# Autodesk Inventor assembly: аккумулятор 18650
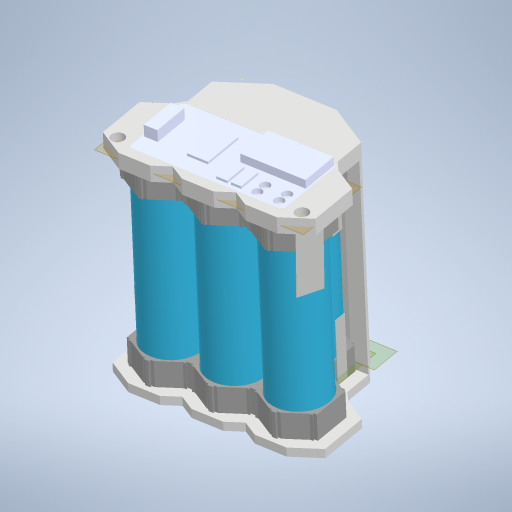
[picture p0: Inventor's stored thumbnail of the model, 512x512]
Saved by Autodesk Inventor 2024.2 (Build 282272000, 272)
## iProperties
Created: 2026-04-21
Part Number: аккумулятор 18650
Document SubType Name: Assembly
Designer: katya_notebook
Author: katya_notebook
## Documents named in this file (12)
- D:\dog\fox\construction\fox\body\аккумулятор 18650.iam
- D:\dog\fox\construction\fox\body\холдерна2.ipt
- D:\dog\fox\construction\fox\body\холдерна3.ipt
- D:\dog\fox\construction\fox\body\18650.ipt
- D:\dog\fox\construction\fox\body\bms\bms.ipt
- D:\dog\fox\construction\fox\body\прямая полоска\прямая полоска.iam
- D:\dog\fox\construction\fox\body\кривая полоска\кривая полоска.iam
- D:\dog\fox\construction\fox\body\кривая полоска тонкая\кривая полоска тонкая.iam
- D:\dog\fox\construction\fox\body\кнопка\кнопка.iam
- D:\dog\fox\construction\fox\body\крепеж.ipt
- D:\dog\fox\construction\fox\body\крепеж бок.ipt
- D:\dog\fox\construction\3dstep\деталька крепление вторая часть.ipt
## Components (24 placed, 11 different names)
1. холдерна2:2 — Жесткий:1, Заподлицо:1, Совмещение:27, Совмещение:29
2. холдерна3:2 — Жесткий:1, Заподлицо:1, Заподлицо:2, С поворотом:3, С поворотом:4, С поворотом:6, Совмещение:7
3. 18650:1 — Заподлицо:2, С поворотом:6, С поворотом:7, Совмещение:8, Совмещение:16
4. 18650:2 — С поворотом:12, С поворотом:16
5. 18650:3 — С поворотом:4, С поворотом:8, Совмещение:6
6. 18650:4 — С поворотом:11, С поворотом:13, С поворотом:14
7. 18650:5 — С поворотом:3, С поворотом:15
8. холдерна2:3 — С поворотом:11, С поворотом:12, Совмещение:3, Совмещение:4, Совмещение:21
9. холдерна3:3 — С поворотом:7, С поворотом:8, Совмещение:3, Совмещение:4, Совмещение:5, Совмещение:15, Совмещение:33, Совмещение:34, Совмещение:35
10. bms:1 — Совмещение:39, Совмещение:40
11. прямая полоска:1 [sub-assembly] — С поворотом:13
12. прямая полоска:2 [sub-assembly] — С поворотом:15, Совмещение:22
13. кривая полоска:1 [sub-assembly] — Совмещение:5, Совмещение:6
14. кривая полоска:2 [sub-assembly] — Совмещение:7, Совмещение:8
15. кривая полоска тонкая:1 [sub-assembly] — Совмещение:21, Совмещение:22
16. кривая полоска тонкая:2 [sub-assembly] — Совмещение:29, Совмещение:30
17. прямая полоска:3 [sub-assembly] — С поворотом:16, Совмещение:28
18. прямая полоска:4 [sub-assembly] — С поворотом:14, Совмещение:30
19. кривая полоска тонкая:3 [sub-assembly] — Совмещение:27, Совмещение:28
20. кривая полоска тонкая:5 [sub-assembly] — Совмещение:15, Совмещение:16
21. кнопка:1 [sub-assembly]
22. крепеж:1 — Совмещение:33, Совмещение:34, Совмещение:35, Совмещение:36, Совмещение:37, Совмещение:38, Совмещение:39, Совмещение:40
23. крепеж бок:1 — Совмещение:36, Совмещение:37, Совмещение:38, Заподлицо:3, Заподлицо:4
24. деталька крепление вторая часть:1 — Заподлицо:3, Заподлицо:4
## Relationships (38: Mate 22, RevoluteJoint 11, Flush 4, WeldJoint 1)
- Жесткий:1 [WeldJoint]: холдерна2:2 ↔ холдерна3:2
- Заподлицо:1 [Flush]: холдерна2:2 ↔ холдерна3:2
- Заподлицо:2 [Flush]: холдерна3:2 ↔ 18650:1
- С поворотом:3 [RevoluteJoint]: холдерна3:2 ↔ 18650:5
- С поворотом:4 [RevoluteJoint]: холдерна3:2 ↔ 18650:3
- С поворотом:6 [RevoluteJoint]: холдерна3:2 ↔ 18650:1
- С поворотом:7 [RevoluteJoint]: 18650:1 ↔ холдерна3:3
- С поворотом:8 [RevoluteJoint]: 18650:3 ↔ холдерна3:3
- С поворотом:11 [RevoluteJoint]: 18650:4 ↔ холдерна2:3
- С поворотом:12 [RevoluteJoint]: 18650:2 ↔ холдерна2:3
- Совмещение:3 [Mate]: холдерна2:3 ↔ холдерна3:3
- Совмещение:4 [Mate]: холдерна2:3 ↔ холдерна3:3
- С поворотом:13 [RevoluteJoint]: 18650:4 ↔ прямая полоска:1
- С поворотом:14 [RevoluteJoint]: 18650:4 ↔ прямая полоска:4
- С поворотом:15 [RevoluteJoint]: 18650:5 ↔ прямая полоска:2
- С поворотом:16 [RevoluteJoint]: 18650:2 ↔ прямая полоска:3
- Совмещение:5 [Mate]: холдерна3:3 ↔ кривая полоска:1
- Совмещение:6 [Mate]: 18650:3 ↔ кривая полоска:1
- Совмещение:7 [Mate]: холдерна3:2 ↔ кривая полоска:2
- Совмещение:8 [Mate]: 18650:1 ↔ кривая полоска:2
- Совмещение:15 [Mate]: холдерна3:3 ↔ кривая полоска тонкая:5
- Совмещение:16 [Mate]: 18650:1 ↔ кривая полоска тонкая:5
- Совмещение:21 [Mate]: холдерна2:3 ↔ кривая полоска тонкая:1
- Совмещение:22 [Mate]: прямая полоска:2 ↔ кривая полоска тонкая:1
- Совмещение:27 [Mate]: холдерна2:2 ↔ кривая полоска тонкая:3
- Совмещение:28 [Mate]: прямая полоска:3 ↔ кривая полоска тонкая:3
- Совмещение:29 [Mate]: холдерна2:2 ↔ кривая полоска тонкая:2
- Совмещение:30 [Mate]: кривая полоска тонкая:2 ↔ прямая полоска:4
- Совмещение:33 [Mate]: холдерна3:3 ↔ крепеж:1
- Совмещение:34 [Mate]: холдерна3:3 ↔ крепеж:1
- Совмещение:35 [Mate]: холдерна3:3 ↔ крепеж:1
- Совмещение:36 [Mate]: крепеж:1 ↔ крепеж бок:1
- Совмещение:37 [Mate]: крепеж:1 ↔ крепеж бок:1
- Совмещение:38 [Mate]: крепеж:1 ↔ крепеж бок:1
- Заподлицо:3 [Flush]: крепеж бок:1 ↔ деталька крепление вторая часть:1
- Заподлицо:4 [Flush]: крепеж бок:1 ↔ деталька крепление вторая часть:1
- Совмещение:39 [Mate]: bms:1 ↔ крепеж:1
- Совмещение:40 [Mate]: bms:1 ↔ крепеж:1
